# Autodesk Inventor assembly: trans-asm-interior
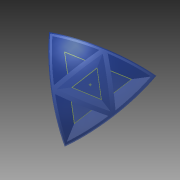
[picture p0: Inventor's stored thumbnail of the model, 180x180]
Saved by Autodesk Inventor 2015 SP2 (Build 190223200, 223)
## iProperties
Created: 2015-05-05
Part Number: trans-asm-interior
Document SubType Name: Assembly
Designer: foote
Mass: 466.005 g
Surface Area: 1246.44 cm^2
Volume: 466.005 cm^3
Density: 1 g/cm^3
Author: foote
## Documents named in this file (4)
- C:\foote\projects\AIR\ommalamp\assembly-2\sect_interior\trans-asm-interior.iam
- C:\foote\projects\AIR\ommalamp\assembly-2\sect_interior\ommatid.ipt
- C:\foote\projects\AIR\ommalamp\assembly-2\sect_interior\ommatid-trans.ipt
- C:\Users\foote\Documents\Inventor\Content Center Files\R2015\en-US\AS 1112 (4)\AS 1112 - M3(2).ipt
## Components (3 placed, 3 different names)
1. ommatid:1 — Mate:12, Angle:3, Mate:14, Mate:15
2. ommatid-trans:1 — Mate:3, Mate:8, Mate:11
3. AS 1112 (4) - Metric M3:3 — Mate:12, Mate:13, Angle:3
## Relationships (8: Mate 7, Angle 1)
- Mate:3: ommatid-trans:1
- Mate:8: ommatid-trans:1
- Mate:11: ommatid-trans:1
- Mate:12 (-0.9017 mm): ommatid:1 ↔ AS 1112 (4) - Metric M3:3
- Mate:13: AS 1112 (4) - Metric M3:3
- Angle:3 (0 deg): ommatid:1 ↔ AS 1112 (4) - Metric M3:3
- Mate:14: ommatid:1
- Mate:15: ommatid:1
## Named parameters: nut_inset = 0.9017 mm, nut_width = 1.8034 mm, magnet_diam = 6.604 mm, magnet_depth = 1.27 mm
